# Autodesk Inventor assembly: Armor_Rear
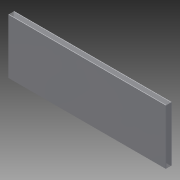
[picture p0: Inventor's stored thumbnail of the model, 180x180]
Saved by Autodesk Inventor 2013 (Build 170138000, 138)
## iProperties
Created: 2015-07-02
Part Number: Armor_Rear
Document SubType Name: Assembly
Designer: Kyle
Mass: 22.0502 g
Surface Area: 259.316 cm^2
Volume: 13.6137 cm^3
Density: 1.6197 g/cm^3
Author: Kyle
## Documents named in this file (3)
- C:\Users\Kyle\Documents\Project documentation\Combat Robot\CAD\V1.0\Armor_Rear.iam
- C:\Users\Kyle\Documents\Project documentation\Combat Robot\CAD\V1.0\Plate_Rear_Poly.ipt
- C:\Users\Kyle\Documents\Project documentation\Combat Robot\CAD\V1.0\Plate_Rear_Alu26.ipt
## Components (3 placed, 2 different names)
1. Plate_Rear_Poly:1 — Mate:1, Flush:1, Flush:2, Mate:2, Flush:3, Flush:4
2. Plate_Rear_Alu26:1 — Mate:1, Flush:1, Flush:2
3. Plate_Rear_Alu26:2 — Mate:2, Flush:3, Flush:4
## Relationships (6: Flush 4, Mate 2)
- Mate:1: Plate_Rear_Poly:1 ↔ Plate_Rear_Alu26:1
- Flush:1: Plate_Rear_Poly:1 ↔ Plate_Rear_Alu26:1
- Flush:2: Plate_Rear_Poly:1 ↔ Plate_Rear_Alu26:1
- Mate:2: Plate_Rear_Poly:1 ↔ Plate_Rear_Alu26:2
- Flush:3: Plate_Rear_Poly:1 ↔ Plate_Rear_Alu26:2
- Flush:4: Plate_Rear_Poly:1 ↔ Plate_Rear_Alu26:2
